# Autodesk Inventor assembly: Assembly
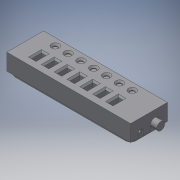
[picture p0: Inventor's stored thumbnail of the model, 180x180]
Saved by Autodesk Inventor 2019 (Build 230136000, 136)
## iProperties
Created: 2019-04-16
Part Number: Assembly
Document SubType Name: Assembly
Designer: zacha
Author: zacha
## Documents named in this file (3)
- H:\Files\Git Repositories\USB Hub Cover\Assembly.iam
- H:\Files\Git Repositories\USB Hub Cover\hub_dummy.ipt
- H:\Files\Git Repositories\USB Hub Cover\cover.ipt
## Components (2 placed, 2 different names)
1. hub_dummy:1 — Flush:1
2. cover:1 — Flush:1
## Relationships (1: Flush 1)
- Flush:1: hub_dummy:1 ↔ cover:1
